# Autodesk Inventor assembly: Assembly_v03
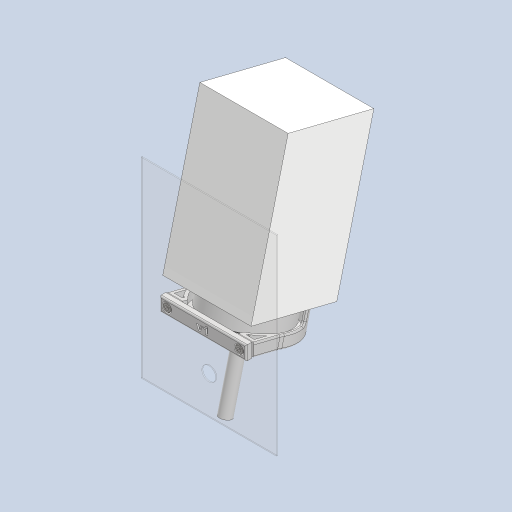
[picture p0: Inventor's stored thumbnail of the model, 512x512]
Saved by Autodesk Inventor 2024.4 (Build 284460000, 460)
## iProperties
Created: 2026-05-05
Part Number: Assembly_v03
Document SubType Name: Assembly
Designer: tooles01
Author: tooles01
## iProperties of the stored document MemberDocs/xW55cntlcN0dy50j2Kcdt4tfrFe
Created: 2026-05-05
Part Number: Assembly_v03
Document SubType Name: Assembly
Designer: tooles01
Author: tooles01
## Documents named in this file (7)
- C:\Users\tooles01\NYU Langone Health Dropbox\Shannon Toole\Shannon_Dropbox\Mar lab\RFID\CAD\Water_bottle\Water_bottle_v03.iam
- C:\Users\tooles01\NYU Langone Health Dropbox\Shannon Toole\Shannon_Dropbox\Mar lab\RFID\CAD\lib\cage_wall_wb.ipt
- C:\Users\tooles01\NYU Langone Health Dropbox\Shannon Toole\Shannon_Dropbox\Mar lab\RFID\CAD\lib\M3 heat-set insert.ipt
- C:\Users\tooles01\Documents\Inventor\Content Center Files\R2024\en-US\AS 1420\AS 1420 - 1973 - M3 x 6.ipt
- C:\Users\tooles01\NYU Langone Health Dropbox\Shannon Toole\Shannon_Dropbox\Mar lab\RFID\CAD\Water_bottle\wb_holder_inside_01.ipt
- C:\Users\tooles01\NYU Langone Health Dropbox\Shannon Toole\Shannon_Dropbox\Mar lab\RFID\CAD\Water_bottle\wb_holder_outside_03.ipt
- C:\Users\tooles01\NYU Langone Health Dropbox\Shannon Toole\Shannon_Dropbox\Mar lab\RFID\CAD\lib\water_bottle_straight.ipt
## Components (8 placed, 6 different names)
1. water_bottle_straight:1 — wall centered to wb, wb to holder, wb to holder base
2. cage_wall_wb:1 — wall centered to wb, holder_outside flush to wall, holder_inside to wall hole:1, holder_inside to wall hole:2
3. wb_holder_outside_03:1 — wb to holder, wb to holder base, holder_outside flush to wall, heat-set to wb holder:1, heat-set to wb holder:2
4. M3 heat-set insert:1 — heat-set to wb holder:1, screw to heat-set:1
5. M3 heat-set insert:2 — heat-set to wb holder:2, screw to heat-set:2
6. AS 1420 - Metric M3 x 6:1 — screw to heat-set:1, screw to inside:1
7. AS 1420 - Metric M3 x 6:2 — screw to heat-set:2, screw to inside:2
8. wb_holder_inside_01:1 — screw to inside:1, screw to inside:2, holder_inside to wall hole:1, holder_inside to wall hole:2
## Relationships (12: Mate 6, Insert 6)
- wall centered to wb [Mate]: water_bottle_straight:1 ↔ cage_wall_wb:1
- wb to holder [Mate]: water_bottle_straight:1 ↔ wb_holder_outside_03:1
- wb to holder base [Mate]: water_bottle_straight:1 ↔ wb_holder_outside_03:1
- heat-set to wb holder:1 [Insert]: wb_holder_outside_03:1 ↔ M3 heat-set insert:1
- heat-set to wb holder:2 [Insert]: wb_holder_outside_03:1 ↔ M3 heat-set insert:2
- screw to inside:1 [Insert]: AS 1420 - Metric M3 x 6:1 ↔ wb_holder_inside_01:1
- screw to inside:2 [Insert]: AS 1420 - Metric M3 x 6:2 ↔ wb_holder_inside_01:1
- screw to heat-set:1 [Mate]: M3 heat-set insert:1 ↔ AS 1420 - Metric M3 x 6:1
- screw to heat-set:2 [Mate]: M3 heat-set insert:2 ↔ AS 1420 - Metric M3 x 6:2
- holder_outside flush to wall [Mate]: cage_wall_wb:1 ↔ wb_holder_outside_03:1
- holder_inside to wall hole:1 [Insert]: cage_wall_wb:1 ↔ wb_holder_inside_01:1
- holder_inside to wall hole:2 [Insert]: cage_wall_wb:1 ↔ wb_holder_inside_01:1
